# Autodesk Inventor assembly: Z belt Sub
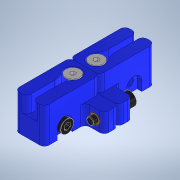
[picture p0: Inventor's stored thumbnail of the model, 180x180]
Saved by Autodesk Inventor 2022 (Build 260153000, 153)
## iProperties
Created: 2022-02-24
Part Number: Z belt Sub
Document SubType Name: Assembly
Designer: Nicoli
Author: Nicoli
## Documents named in this file (6)
- Y:\Projects\Bibble0\SubAsm\Z belt Sub.iam
- Y:\Projects\Bibble0\3D printed\Z Axis\Z Belt Clip with HSI.iam
- Y:\Projects\Bibble0\3D printed\Z Axis\Z Belt Housing HSI.iam
- Y:\Projects\Bibble0\Hardware\M3 x 14 mm  SHCS.ipt
- Y:\Projects\Bibble0\3D printed\Z Axis\Z Belt Tensioner - Mirror HSI.iam
- Y:\Projects\Bibble0\Hardware\M3 x 10 mm FHCS.ipt
## Components (7 placed, 5 different names)
1. Z Belt Clip with HSI:1 [sub-assembly] — Insert:1, Insert:3, Insert:4, Flush:1, Flush:2, Mate:2
2. Z Belt Housing HSI:1 [sub-assembly] — Insert:1, Angle:1
3. M3 x 14 mm  SHCS:1 — Insert:3
4. Z Belt Tensioner - Mirror HSI:1 [sub-assembly] — Insert:4, Flush:1, Angle:1, Flush:3, Mate:1, Insert:5
5. M3 x 10 mm FHCS:1 — Flush:2, Mate:2
6. M3 x 10 mm FHCS:2 — Flush:3, Mate:1
7. M3 x 14 mm  SHCS:2 — Insert:5
## Relationships (10: Insert 4, Flush 3, Mate 2, Angle 1)
- Insert:1 (0.2 mm): Z Belt Clip with HSI:1 ↔ Z Belt Housing HSI:1
- Insert:3: Z Belt Clip with HSI:1 ↔ M3 x 14 mm  SHCS:1
- Insert:4: Z Belt Clip with HSI:1 ↔ Z Belt Tensioner - Mirror HSI:1
- Flush:1: Z Belt Clip with HSI:1 ↔ Z Belt Tensioner - Mirror HSI:1
- Angle:1 (0 deg): Z Belt Housing HSI:1 ↔ Z Belt Tensioner - Mirror HSI:1
- Flush:2: Z Belt Clip with HSI:1 ↔ M3 x 10 mm FHCS:1
- Flush:3: Z Belt Tensioner - Mirror HSI:1 ↔ M3 x 10 mm FHCS:2
- Mate:1: Z Belt Tensioner - Mirror HSI:1 ↔ M3 x 10 mm FHCS:2
- Mate:2: Z Belt Clip with HSI:1 ↔ M3 x 10 mm FHCS:1
- Insert:5: Z Belt Tensioner - Mirror HSI:1 ↔ M3 x 14 mm  SHCS:2
